# Autodesk Inventor assembly: Locker Assembly
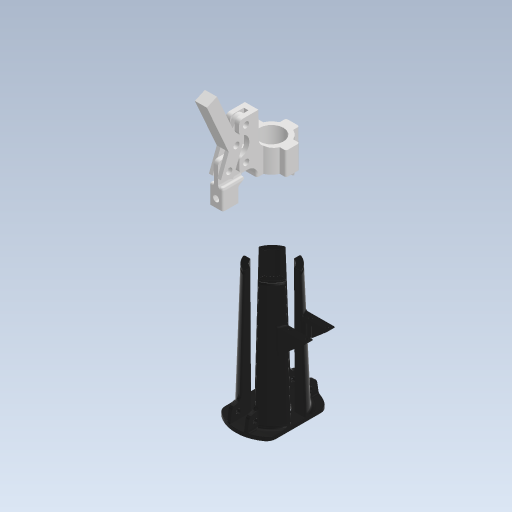
[picture p0: Inventor's stored thumbnail of the model, 512x512]
Saved by Autodesk Inventor 2023 (Build 270158000, 158)
## iProperties
Created: 2022-09-16
Part Number: Locker Assembly
Document SubType Name: Assembly
Designer: Dave
Author: Dave
## Documents named in this file (6)
- C:\Users\Dave\Documents\GrabCAD\Chalk Bot\Chalkbot1.0\Apparatus\V3.2\Locker Assembly.iam
- C:\Users\Dave\Documents\GrabCAD\Chalk Bot\Chalkbot1.0\Apparatus\V3.2\R2.ipt
- C:\Users\Dave\Documents\GrabCAD\Chalk Bot\Chalkbot1.0\Apparatus\V3.2\R3.ipt
- C:\Users\Dave\Documents\GrabCAD\Chalk Bot\Chalkbot1.0\Apparatus\V3.2\r4.ipt
- C:\Users\Dave\Documents\GrabCAD\Chalk Bot\Chalkbot1.0\Apparatus\V3.2\Slider.ipt
- C:\Users\Dave\Documents\GrabCAD\Chalk Bot\Chalkbot1.0\Apparatus\V3\Apparatus Collet V6 CF Springs.ipt
## Components (5 placed, 5 different names)
1. R2:1 — Mate:1, Mate:2, Mate:3
2. R3:1 — Insert:1, Mate:2
3. r4:1 — Insert:3, Mate:1, Mate:3, Angle:1
4. Slider:1 — Insert:1, Insert:3, Angle:1, Mate:4, Angle:2
5. Apparatus Collet V6 CF Springs:1 — Mate:4, Angle:2
## Relationships (8: Mate 4, Insert 2, Angle 2)
- Insert:1: R3:1 ↔ Slider:1
- Insert:3: r4:1 ↔ Slider:1
- Mate:1: R2:1 ↔ r4:1
- Mate:2: R2:1 ↔ R3:1
- Mate:3: R2:1 ↔ r4:1
- Angle:1 (0 deg): r4:1 ↔ Slider:1
- Mate:4: Slider:1 ↔ Apparatus Collet V6 CF Springs:1
- Angle:2 (0 deg): Slider:1 ↔ Apparatus Collet V6 CF Springs:1
